# Autodesk Inventor assembly: motor_mount
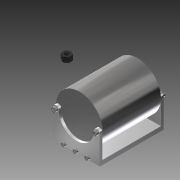
[picture p0: Inventor's stored thumbnail of the model, 180x180]
Saved by Autodesk Inventor 2019 (Build 230136000, 136)
## iProperties
Created: 2018-09-24
Part Number: motor_mount
Document SubType Name: Assembly
Designer: Callum Snowden
Mass: 10252.9 g
Surface Area: 1329.7 cm^2
Volume: 1436.08 cm^3
Density: 7.13948 g/cm^3
Author: Callum Snowden
## Documents named in this file (12)
- C:\Users\Callum\Documents\GitHub\clasohlsonkart\mechanical\motor\motor_mount.iam
- C:\Users\Callum\Documents\GitHub\clasohlsonkart\mechanical\motor\boma_2kw_motor.ipt
- C:\Users\Callum\Documents\GitHub\clasohlsonkart\mechanical\motor\motor_end_plate.ipt
- C:\Users\Callum\Documents\GitHub\clasohlsonkart\mechanical\motor\motor_base_plate.ipt
- C:\Users\Callum\Documents\Inventor\Content Center Files\R2019\en-US\BS 4320(2)\BS 4320 - M6 (Form B).ipt
- C:\Users\Callum\Documents\Inventor\Content Center Files\R2019\en-US\BS 4168(1)\BS 4168 - M6 x 16(1).ipt
- C:\Users\Callum\Documents\Inventor\Content Center Files\R2019\en-US\BS 4168(1)\BS 4168 - M5 x 16(1).ipt
- C:\Users\Callum\Documents\Inventor\Content Center Files\R2019\en-US\BS EN 24034\ISO 4034 - M12BS EN.ipt
- C:\Users\Callum\Documents\GitHub\clasohlsonkart\mechanical\motor\motor_mount\AIP\FEA\cn71sb4o0.fins
- C:\Users\Callum\Documents\GitHub\clasohlsonkart\mechanical\motor\motor_mount\AIP\FEA\cn71sb4o0.fsat
- C:\Users\Callum\Documents\GitHub\clasohlsonkart\mechanical\motor\motor_mount\AIP\FEA\cn71sb4o0.ftes
- C:\Users\Callum\Documents\GitHub\clasohlsonkart\mechanical\motor\motor_mount\AIP\FEA\cn71sb4o0.fwiz
## Components (17 placed, 7 different names)
1. boma_2kw_motor:1 — Rigid:1
2. motor_end_plate:1 — Rigid:1, Rigid:2, Insert:3, Insert:4, Insert:8, Insert:9, Insert:10
3. motor_end_plate:2 — Rigid:3, Rigid:4, Rigid:5, Insert:1, Insert:2, Insert:5, Insert:6, Insert:7
4. motor_base_plate:1 — Rigid:2, Rigid:3
5. BS 4320 Form AB M6 (Form B):1 — Rigid:5
6. BS 4320 Form AB M6 (Form B):2 — Rigid:4
7. BS 4168 : Part 1 Hexagon Socket Head Cap Screw - Metric M6 x 16:1 — Insert:2
8. BS 4168 : Part 1 Hexagon Socket Head Cap Screw - Metric M6 x 16:2 — Insert:1
9. BS 4168 : Part 1 Hexagon Socket Head Cap Screw - Metric M6 x 16:3 — Insert:3
10. BS 4168 : Part 1 Hexagon Socket Head Cap Screw - Metric M6 x 16:4 — Insert:4
11. BS 4168 : Part 1 Hexagon Socket Head Cap Screw - Metric M5 x 16:1 — Insert:5
12. BS 4168 : Part 1 Hexagon Socket Head Cap Screw - Metric M5 x 16:2 — Insert:6
13. BS 4168 : Part 1 Hexagon Socket Head Cap Screw - Metric M5 x 16:3 — Insert:7
14. BS 4168 : Part 1 Hexagon Socket Head Cap Screw - Metric M5 x 16:4 — Insert:8
15. BS 4168 : Part 1 Hexagon Socket Head Cap Screw - Metric M5 x 16:5 — Insert:9
16. BS 4168 : Part 1 Hexagon Socket Head Cap Screw - Metric M5 x 16:6 — Insert:10
17. BS EN 24034 - Metric M12:1
## Relationships (15: Insert 10, WeldJoint 5)
- Rigid:1 [WeldJoint]: boma_2kw_motor:1 ↔ motor_end_plate:1
- Rigid:2 [WeldJoint]: motor_end_plate:1 ↔ motor_base_plate:1
- Rigid:3 [WeldJoint]: motor_end_plate:2 ↔ motor_base_plate:1
- Rigid:4 [WeldJoint]: motor_end_plate:2 ↔ BS 4320 Form AB M6 (Form B):2
- Rigid:5 [WeldJoint]: motor_end_plate:2 ↔ BS 4320 Form AB M6 (Form B):1
- Insert:1: motor_end_plate:2 ↔ BS 4168 : Part 1 Hexagon Socket Head Cap Screw - Metric M6 x 16:2
- Insert:2: motor_end_plate:2 ↔ BS 4168 : Part 1 Hexagon Socket Head Cap Screw - Metric M6 x 16:1
- Insert:3: motor_end_plate:1 ↔ BS 4168 : Part 1 Hexagon Socket Head Cap Screw - Metric M6 x 16:3
- Insert:4: motor_end_plate:1 ↔ BS 4168 : Part 1 Hexagon Socket Head Cap Screw - Metric M6 x 16:4
- Insert:5: motor_end_plate:2 ↔ BS 4168 : Part 1 Hexagon Socket Head Cap Screw - Metric M5 x 16:1
- Insert:6: motor_end_plate:2 ↔ BS 4168 : Part 1 Hexagon Socket Head Cap Screw - Metric M5 x 16:2
- Insert:7: motor_end_plate:2 ↔ BS 4168 : Part 1 Hexagon Socket Head Cap Screw - Metric M5 x 16:3
- Insert:8: motor_end_plate:1 ↔ BS 4168 : Part 1 Hexagon Socket Head Cap Screw - Metric M5 x 16:4
- Insert:9: motor_end_plate:1 ↔ BS 4168 : Part 1 Hexagon Socket Head Cap Screw - Metric M5 x 16:5
- Insert:10: motor_end_plate:1 ↔ BS 4168 : Part 1 Hexagon Socket Head Cap Screw - Metric M5 x 16:6
